# Autodesk Inventor assembly: stand
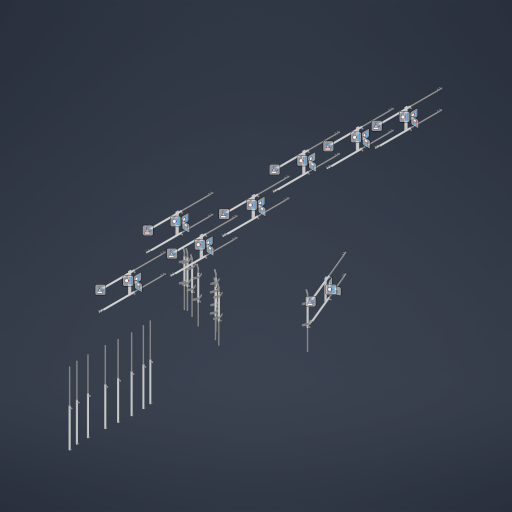
[picture p0: Inventor's stored thumbnail of the model, 512x512]
Saved by Autodesk Inventor 2023 (Build 270158000, 158)
## iProperties
Created: 2022-04-27
Part Number: stand
Document SubType Name: Assembly
Designer: Norbert Ligas
Author: Norbert Ligas
## Documents named in this file (4)
- C:\Users\norbe\Repozytoria\NormalMapScanner\stand_construction\stand.iam
- C:\Users\norbe\Repozytoria\NormalMapScanner\stand_construction\parts\adjustable_leg.iam
- C:\Users\norbe\Repozytoria\NormalMapScanner\stand_construction\parts\adjustable_double_connector.iam
- C:\Users\norbe\Repozytoria\NormalMapScanner\stand_construction\parts\adjustable_arm.iam
## Components (24 placed, 3 different names)
1. adjustable_leg:1 [sub-assembly] — Mate:1, Flush:1, Flush:2, Flush:3, Tangent:1, Mate:4, Mate:5
2. adjustable_leg:2 [sub-assembly]
3. adjustable_leg:3 [sub-assembly]
4. adjustable_leg:4 [sub-assembly]
5. adjustable_leg:5 [sub-assembly]
6. adjustable_leg:6 [sub-assembly]
7. adjustable_leg:7 [sub-assembly]
8. adjustable_leg:8 [sub-assembly]
9. adjustable_double_connector:1 [sub-assembly]
10. adjustable_double_connector:2 [sub-assembly]
11. adjustable_double_connector:3 [sub-assembly]
12. adjustable_double_connector:4 [sub-assembly]
13. adjustable_double_connector:5 [sub-assembly]
14. adjustable_double_connector:6 [sub-assembly]
15. adjustable_double_connector:7 [sub-assembly]
16. adjustable_double_connector:8 [sub-assembly] — Tangent:1, Mate:4, Mate:5
17. adjustable_arm:1 [sub-assembly]
18. adjustable_arm:2 [sub-assembly]
19. adjustable_arm:3 [sub-assembly]
20. adjustable_arm:4 [sub-assembly]
21. adjustable_arm:5 [sub-assembly]
22. adjustable_arm:6 [sub-assembly]
23. adjustable_arm:7 [sub-assembly]
24. adjustable_arm:8 [sub-assembly]
## Relationships (7: Mate 3, Flush 3, Tangent 1)
- Mate:1: adjustable_leg:1
- Flush:1: adjustable_leg:1
- Flush:2: adjustable_leg:1
- Flush:3: adjustable_leg:1
- Tangent:1: adjustable_leg:1 ↔ adjustable_double_connector:8
- Mate:4: adjustable_leg:1 ↔ adjustable_double_connector:8
- Mate:5: adjustable_leg:1 ↔ adjustable_double_connector:8
## Named parameters: arm_min_length = 300 mm, arm_max_length = 565 mm, max_extrusion = 265 mm, min_extrusion = 0 mm, hinge_insertion = 15 mm, connection_length = 20 mm, bar_length = 285 mm, pipe_length = 300 mm
